# Autodesk Inventor assembly: RobotPallet_2
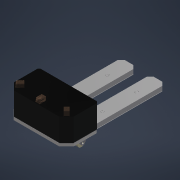
[picture p0: Inventor's stored thumbnail of the model, 180x180]
Saved by Autodesk Inventor 2022 (Build 260153000, 153)
## iProperties
Created: 2021-09-10
Part Number: RobotPallet_2
Material: Generic
Document SubType Name: Assembly
Designer: Andres
Author: Andres
## Documents named in this file (11)
- D:\Documentos\15.PUCP_2021-2\[PDM] Proyecto de Diseño Mecatrónico\ProyectoGIT\ProyectoRobotPallet\RobotPallet_2.iam
- D:\Documentos\15.PUCP_2021-2\[PDM] Proyecto de Diseño Mecatrónico\ProyectoGIT\ProyectoRobotPallet\Estructura Inferior.iam
- D:\Documentos\15.PUCP_2021-2\[PDM] Proyecto de Diseño Mecatrónico\ProyectoGIT\ProyectoRobotPallet\plancah base.ipt
- D:\Documentos\15.PUCP_2021-2\[PDM] Proyecto de Diseño Mecatrónico\ProyectoGIT\ProyectoRobotPallet\apoyo\apoyo2.ipt
- D:\Documentos\15.PUCP_2021-2\[PDM] Proyecto de Diseño Mecatrónico\ProyectoGIT\ProyectoRobotPallet\Mecanismo de movimiento\Mecanismo - Izquierdo.iam
- D:\Documentos\15.PUCP_2021-2\[PDM] Proyecto de Diseño Mecatrónico\ProyectoGIT\ProyectoRobotPallet\Mecanismo de movimiento\Mecanismo - Derecho.iam
- D:\Documentos\15.PUCP_2021-2\[PDM] Proyecto de Diseño Mecatrónico\ProyectoGIT\ProyectoRobotPallet\Horquillas\Horquilla.iam
- D:\Documentos\15.PUCP_2021-2\[PDM] Proyecto de Diseño Mecatrónico\ProyectoGIT\ProyectoRobotPallet\Carcasa.ipt
- D:\Documentos\15.PUCP_2021-2\[PDM] Proyecto de Diseño Mecatrónico\ProyectoGIT\ProyectoRobotPallet\LIDARLivox Mid-70.ipt
- D:\Documentos\15.PUCP_2021-2\[PDM] Proyecto de Diseño Mecatrónico\ProyectoGIT\ProyectoRobotPallet\Bateria de camion.ipt
- D:\Documentos\15.PUCP_2021-2\[PDM] Proyecto de Diseño Mecatrónico\ProyectoGIT\ProyectoRobotPallet\Intel_RealSense_Depth_Camera_D435.ipt
## Components (16 placed, 10 different names)
1. Estructura Inferior:1 [sub-assembly] — Flush:1, Coincidencia:1, Coincidencia:2, Coincidencia:3, Coincidencia:4, Coincidencia:6, Coincidencia:8, Nivelación:3, Nivelación:4, Nivelación:5, Nivelación:6, Coincidencia:9, Coincidencia:10, Coincidencia:11, Coincidencia:12, Coincidencia:13, Coincidencia:14, Ángulo:1, Ángulo:2, Nivelación:14, Nivelación:15, Nivelación:16
2. planchabase:1 — Flush:1, Nivelación:2, Nivelación:7, Nivelación:8, Nivelación:14, Nivelación:15, Nivelación:16, Coincidencia:22
3. apoyo2:1 — Coincidencia:1, Nivelación:5
4. apoyo2:2 — Coincidencia:2, Coincidencia:5, Nivelación:6
5. apoyo2:3 — Coincidencia:3, Nivelación:4
6. apoyo2:4 — Coincidencia:4, Coincidencia:7, Nivelación:3
7. Mecanismo - Izquierdo:1 [sub-assembly] — Coincidencia:5, Coincidencia:6, Ángulo:2
8. Mecanismo - Derecho:1 [sub-assembly] — Coincidencia:7, Coincidencia:8, Ángulo:1
9. Horquilla:1 [sub-assembly] — Coincidencia:9, Coincidencia:11, Coincidencia:13
10. Horquilla:2 [sub-assembly] — Coincidencia:10, Coincidencia:12, Coincidencia:14
11. Carcasa:1 — Nivelación:7, Nivelación:8, Coincidencia:22, Mate:23, Mate:24, Mate:25, Flush:17, Flush:18, Flush:19, Mate:26
12. LIDARLivox Mid-70:1 — Mate:24, Flush:18
13. LIDARLivox Mid-70:2 — Mate:25, Flush:17
14. LIDARLivox Mid-70:3 — Mate:23, Flush:19
15. Bateria de camion:1
16. Intel_RealSense_Depth_Camera_D435:1 — Mate:26
## Relationships (35: Mate 19, Flush 14, Angle 2)
- Flush:1: Estructura Inferior:1 ↔ planchabase:1
- Nivelación:2 [Flush]: planchabase:1
- Coincidencia:1 [Mate]: Estructura Inferior:1 ↔ apoyo2:1
- Coincidencia:2 [Mate]: Estructura Inferior:1 ↔ apoyo2:2
- Coincidencia:3 [Mate]: Estructura Inferior:1 ↔ apoyo2:3
- Coincidencia:4 [Mate]: Estructura Inferior:1 ↔ apoyo2:4
- Coincidencia:5 [Mate]: apoyo2:2 ↔ Mecanismo - Izquierdo:1
- Coincidencia:6 [Mate] (2.5 mm): Estructura Inferior:1 ↔ Mecanismo - Izquierdo:1
- Coincidencia:7 [Mate]: apoyo2:4 ↔ Mecanismo - Derecho:1
- Coincidencia:8 [Mate] (2.5 mm): Estructura Inferior:1 ↔ Mecanismo - Derecho:1
- Nivelación:3 [Flush] (180 mm): Estructura Inferior:1 ↔ apoyo2:4
- Nivelación:4 [Flush] (180 mm): Estructura Inferior:1 ↔ apoyo2:3
- Nivelación:5 [Flush] (180 mm): Estructura Inferior:1 ↔ apoyo2:1
- Nivelación:6 [Flush] (180 mm): Estructura Inferior:1 ↔ apoyo2:2
- Coincidencia:9 [Mate]: Estructura Inferior:1 ↔ Horquilla:1
- Coincidencia:10 [Mate]: Estructura Inferior:1 ↔ Horquilla:2
- Coincidencia:11 [Mate]: Estructura Inferior:1 ↔ Horquilla:1
- Coincidencia:12 [Mate]: Estructura Inferior:1 ↔ Horquilla:2
- Coincidencia:13 [Mate] (-110 mm): Estructura Inferior:1 ↔ Horquilla:1
- Coincidencia:14 [Mate] (-110 mm): Estructura Inferior:1 ↔ Horquilla:2
- Ángulo:1 [Angle] (0 deg): Estructura Inferior:1 ↔ Mecanismo - Derecho:1
- Ángulo:2 [Angle] (180 deg): Estructura Inferior:1 ↔ Mecanismo - Izquierdo:1
- Nivelación:7 [Flush]: planchabase:1 ↔ Carcasa:1
- Nivelación:8 [Flush]: planchabase:1 ↔ Carcasa:1
- Nivelación:14 [Flush] (4 mm): Estructura Inferior:1 ↔ planchabase:1
- Nivelación:15 [Flush] (-4 mm): Estructura Inferior:1 ↔ planchabase:1
- Nivelación:16 [Flush] (-4 mm): Estructura Inferior:1 ↔ planchabase:1
- Coincidencia:22 [Mate]: planchabase:1 ↔ Carcasa:1
- Mate:23 (-10 mm): Carcasa:1 ↔ LIDARLivox Mid-70:3
- Mate:24 (-10 mm): Carcasa:1 ↔ LIDARLivox Mid-70:1
- Mate:25 (-10 mm): Carcasa:1 ↔ LIDARLivox Mid-70:2
- Flush:17 (10 mm): Carcasa:1 ↔ LIDARLivox Mid-70:2
- Flush:18 (10 mm): Carcasa:1 ↔ LIDARLivox Mid-70:1
- Flush:19 (10 mm): Carcasa:1 ↔ LIDARLivox Mid-70:3
- Mate:26 (-20 mm): Carcasa:1 ↔ Intel_RealSense_Depth_Camera_D435:1
